# Autodesk Inventor assembly: assembly_gripper
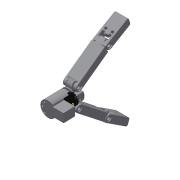
[picture p0: Inventor's stored thumbnail of the model, 180x180]
Saved by Autodesk Inventor 2018 (Build 220112000, 112)
## iProperties
Created: 2018-04-13
Part Number: assembly_gripper
Material: Genérico
Document SubType Name: Assembly
Designer: se_ma
Author: se_ma
## Documents named in this file (8)
- E:\programming\hecatonquiros\cad_models\tools\gripper\two_fingers_tensor\assembly_gripper.iam
- E:\programming\hecatonquiros\cad_models\tools\gripper\two_fingers_tensor\base.ipt
- E:\programming\hecatonquiros\cad_models\tools\gripper\two_fingers_tensor\finger_long.ipt
- E:\programming\hecatonquiros\cad_models\tools\gripper\two_fingers_tensor\finger_short.ipt
- E:\programming\hecatonquiros\cad_models\tools\gripper\two_fingers_tensor\enganche_servo.ipt
- E:\programming\hecatonquiros\cad_models\tools\gripper\two_fingers_tensor\eng_chic_2_1.ipt
- E:\programming\hecatonquiros\cad_models\tools\gripper\two_fingers_tensor\eng_gran_2_1.ipt
- E:\programming\hecatonquiros\cad_models\tools\gripper\two_fingers_tensor\microservo_FT.ipt
## Components (9 placed, 7 different names)
1. base:1 — Coincidencia:1, Coincidencia:2, Coincidencia:3, Coincidencia:4, Mate:9, Mate:10, Mate:13, Mate:14
2. finger_long:1 — Coincidencia:1, Coincidencia:2, Coincidencia:7, Coincidencia:8
3. finger_long:2 — Coincidencia:3, Coincidencia:4, Coincidencia:5, Coincidencia:6
4. finger_short:1 — Coincidencia:5, Coincidencia:6
5. finger_short:2 — Coincidencia:7, Coincidencia:8
6. enganche_servo:1 — Mate:9, Mate:10, Mate:15
7. eng_chic_2_1:1 — Mate:13, Mate:14, Flush:1
8. eng_gran_2_1:1 — Flush:1
9. microservo_FT:1 — Mate:15
## Relationships (14: Mate 13, Flush 1)
- Coincidencia:1 [Mate]: base:1 ↔ finger_long:1
- Coincidencia:2 [Mate]: base:1 ↔ finger_long:1
- Coincidencia:3 [Mate]: base:1 ↔ finger_long:2
- Coincidencia:4 [Mate]: base:1 ↔ finger_long:2
- Coincidencia:5 [Mate]: finger_long:2 ↔ finger_short:1
- Coincidencia:6 [Mate]: finger_long:2 ↔ finger_short:1
- Coincidencia:7 [Mate]: finger_long:1 ↔ finger_short:2
- Coincidencia:8 [Mate]: finger_long:1 ↔ finger_short:2
- Mate:9: base:1 ↔ enganche_servo:1
- Mate:10: base:1 ↔ enganche_servo:1
- Mate:13: base:1 ↔ eng_chic_2_1:1
- Mate:14: base:1 ↔ eng_chic_2_1:1
- Flush:1: eng_chic_2_1:1 ↔ eng_gran_2_1:1
- Mate:15: enganche_servo:1 ↔ microservo_FT:1
